# Autodesk Inventor assembly: EnsamblajeBarco
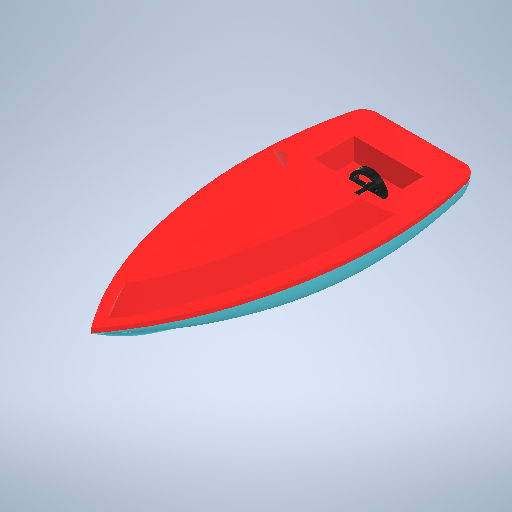
[picture p0: Inventor's stored thumbnail of the model, 512x512]
Saved by Autodesk Inventor 2025.2 (Build 292293000, 293)
## iProperties
Created: 2025-01-18
Part Number: EnsamblajeBarco
Document SubType Name: Assembly
Designer: usuario
Author: usuario
## Documents named in this file (4)
- C:\Users\usuario\Desktop\EnsamblajeBarco.iam
- C:\Users\usuario\Desktop\PiezabarcoInferior.ipt
- C:\Users\usuario\Desktop\Piezabarcosuperior.ipt
- C:\Users\usuario\Desktop\PiezaTimon.ipt
## Components (3 placed, 3 different names)
1. PiezabarcoInferior:1 — Coincidencia:1, Nivelación:1, Coincidencia:2
2. Piezabarcosuperior:1 — Coincidencia:1, Nivelación:1, Coincidencia:2, Coincidencia:3, Coincidencia:4
3. PiezaTimon:1 — Coincidencia:3, Coincidencia:4
## Relationships (5: Mate 4, Flush 1)
- Coincidencia:1 [Mate]: PiezabarcoInferior:1 ↔ Piezabarcosuperior:1
- Nivelación:1 [Flush]: PiezabarcoInferior:1 ↔ Piezabarcosuperior:1
- Coincidencia:2 [Mate]: PiezabarcoInferior:1 ↔ Piezabarcosuperior:1
- Coincidencia:3 [Mate]: Piezabarcosuperior:1 ↔ PiezaTimon:1
- Coincidencia:4 [Mate]: Piezabarcosuperior:1 ↔ PiezaTimon:1
